# Autodesk Inventor assembly: Assembly9
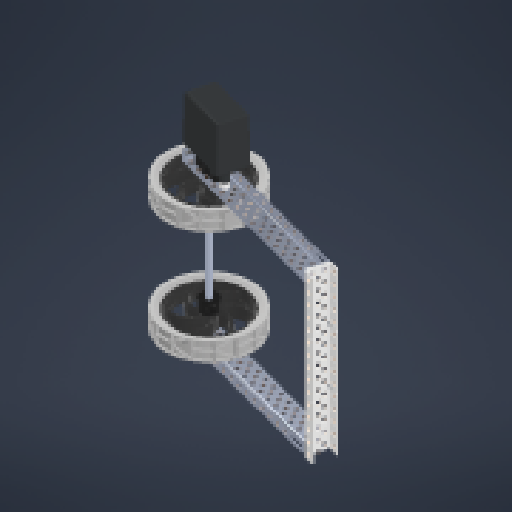
[picture p0: Inventor's stored thumbnail of the model, 512x512]
Saved by Autodesk Inventor 2023 (Build 270158000, 158)
## iProperties
Created: 2023-02-06
Part Number: Assembly9
Document SubType Name: Assembly
Designer: Windows Macbook
Author: Windows Macbook
## Documents named in this file (14)
- C:\Users\Windows Macbook\Desktop\Inventor\Assembly9.iam
- C:\Users\Windows Macbook\Documents\Inventor\Content Center Files\VEX-CAD-Inventor-1.4.0\Structure\Chassis Rails\Steel Chassis Rail 2x1x16.ipt
- C:\Users\Windows Macbook\Documents\Inventor\Content Center Files\VEX-CAD-Inventor-1.4.0\Motion\Shaft HS\HS Bearing Flat.ipt
- C:\Users\Windows Macbook\Documents\Inventor\Content Center Files\VEX-CAD-Inventor-1.4.0\Motion\Shaft HS\HS Shaft Collar.ipt
- C:\Users\Windows Macbook\Documents\Inventor\Content Center Files\VEX-CAD-Inventor-1.4.0\Motion\Shaft HS\Shaft HS\Shaft HS 8.0 in.ipt
- C:\Users\Windows Macbook\Documents\Inventor\Content Center Files\VEX-CAD-Inventor-1.4.0\Motion\Shaft HS\Shaft HS.ipt
- C:\Users\Windows Macbook\Documents\Inventor\Content Center Files\VEX-CAD-Inventor-1.4.0\Structure\C Channel\Aluminum 1x2x1\Alu C 1x2x1x15.ipt
- C:\Users\Windows Macbook\Documents\Inventor\Content Center Files\VEX-CAD-Inventor-1.4.0\Motion\Wheels\Traction Wheel.iam
- C:\Users\Windows Macbook\Documents\Inventor\Content Center Files\VEX-CAD-Inventor-1.4.0\Motion\Wheels\Traction Wheel\4 Traction, No Insert.iam
- C:\Users\Windows Macbook\Documents\Inventor\Content Center Files\VEX-CAD-Inventor-1.4.0\Motion\Shaft HS\HS Spacer.ipt
- C:\Users\Windows Macbook\Documents\Inventor\Content Center Files\VEX-CAD-Inventor-1.4.0\Motion\Shaft HS\HS Spacer\HSpacer .2500.ipt
- C:\Users\Windows Macbook\Documents\Inventor\Content Center Files\VEX-CAD-Inventor-1.4.0\Motion\Spacers\Spacer Nylon .313 OD\NSpacer .313 OD x .250.ipt
- C:\Users\Windows Macbook\Documents\Inventor\Content Center Files\VEX-CAD-Inventor-1.4.0\Motion\Spacers\Spacer Nylon .313 OD.ipt
- C:\Users\Windows Macbook\Documents\Inventor\Content Center Files\VEX-CAD-Inventor-1.4.0\Electronics\V5 Simple Motor.ipt
## Components (15 placed, 9 different names)
1. Alu C 1x2x1x15:1 — Flush:7
2. Steel Chassis Rail 2x1x16:1 — Insert:9, Insert:10, Insert:11, Insert:17
3. Steel Chassis Rail 2x1x16:2 — Insert:7, Insert:8, Flush:7, Insert:14
4. HS Bearing Flat:1 — Insert:9, Insert:10, Insert:18
5. HS Bearing Flat:2 — Insert:6, Insert:7, Insert:8
6. HS Shaft Collar:1 — Insert:6, Flush:6, Cylindrical:1
7. Shaft HS 8.0 in:1 — Flush:6, Cylindrical:1
8. 4 Traction, No Insert:1 [sub-assembly] — Insert:12, Insert:15
9. HSpacer .2500:1 — Insert:11, Insert:12
10. 4 Traction, No Insert:2 [sub-assembly] — Insert:16
11. HSpacer .2500:2 — Insert:14
12. HS Shaft Collar:3 — Insert:15
13. HS Shaft Collar:4 — Insert:16
14. NSpacer .313 OD x .250:1 — Insert:17, Insert:19
15. V5 Simple Motor:1 — Insert:18, Insert:19
## Relationships (22: Insert 14, Flush 5, Mate 2, CylindricalJoint 1)
- [Flush]: Alu C 1x2x1x15:1 ↔ Steel Chassis Rail 2x1x16:1
- [Mate]: Alu C 1x2x1x15:1 ↔ Steel Chassis Rail 2x1x16:1
- [Flush]: Alu C 1x2x1x15:1 ↔ Steel Chassis Rail 2x1x16:1
- [Mate]: Alu C 1x2x1x15:1 ↔ Steel Chassis Rail 2x1x16:2
- [Flush]: Alu C 1x2x1x15:1 ↔ Steel Chassis Rail 2x1x16:2
- Insert:6: HS Bearing Flat:2 ↔ HS Shaft Collar:1
- Insert:7: Steel Chassis Rail 2x1x16:2 ↔ HS Bearing Flat:2
- Insert:8: Steel Chassis Rail 2x1x16:2 ↔ HS Bearing Flat:2
- Flush:6 (-3.175 mm): HS Shaft Collar:1 ↔ Shaft HS 8.0 in:1
- Cylindrical:1: HS Shaft Collar:1 ↔ Shaft HS 8.0 in:1
- Flush:7: Alu C 1x2x1x15:1 ↔ Steel Chassis Rail 2x1x16:2
- Insert:9: Steel Chassis Rail 2x1x16:1 ↔ HS Bearing Flat:1
- Insert:10: Steel Chassis Rail 2x1x16:1 ↔ HS Bearing Flat:1
- Insert:11: Steel Chassis Rail 2x1x16:1 ↔ HSpacer .2500:1
- Insert:12: 4 Traction, No Insert:1 ↔ HSpacer .2500:1
- [Insert]: 4 Traction, No Insert:2 ↔ HSpacer .2500:2
- Insert:14: Steel Chassis Rail 2x1x16:2 ↔ HSpacer .2500:2
- Insert:15: 4 Traction, No Insert:1 ↔ HS Shaft Collar:3
- Insert:16: 4 Traction, No Insert:2 ↔ HS Shaft Collar:4
- Insert:17: Steel Chassis Rail 2x1x16:1 ↔ NSpacer .313 OD x .250:1
- Insert:18: HS Bearing Flat:1 ↔ V5 Simple Motor:1
- Insert:19 (1.6221 mm): NSpacer .313 OD x .250:1 ↔ V5 Simple Motor:1
## Named parameters: d24_d23 = 0 mm
